# Autodesk Inventor assembly: ensamble taza simpson
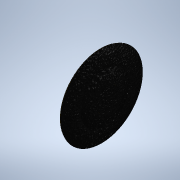
[picture p0: Inventor's stored thumbnail of the model, 180x180]
Saved by Autodesk Inventor 2021 (Build 250183000, 183)
## iProperties
Created: 2021-07-02
Part Number: ensamble taza simpson
Document SubType Name: Assembly
Designer: uriel
Author: uriel
## Documents named in this file (3)
- C:\Users\uriel\OneDrive\Documentos\ensamble taza simpson.iam
- C:\Users\uriel\OneDrive\Documentos\taza.ipt
- C:\Users\uriel\OneDrive\Documentos\plato.ipt
## Components (2 placed, 2 different names)
1. taza:1 — De rotación:1
2. plato:1 — De rotación:1
## Relationships (1: RevoluteJoint 1)
- De rotación:1 [RevoluteJoint]: taza:1 ↔ plato:1
